# Autodesk Inventor assembly: Full overlay hinge for aluminium frame
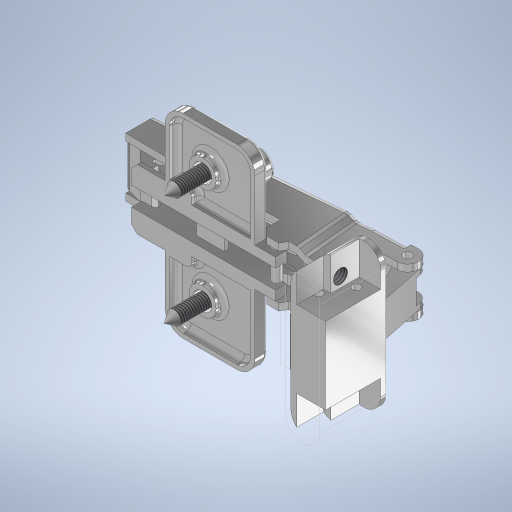
[picture p0: Inventor's stored thumbnail of the model, 512x512]
Saved by Autodesk Inventor 2024 (Build 280153000, 153)
## iProperties
Created: 2014-01-06
Part Number: Full overlay hinge for aluminium frame
Document SubType Name: Assembly
Designer: G. Kazokaitis
Author: G. Kazokaitis
## Documents named in this file (15)
- C:\W4INV 2024 Design\LIBRARY\Hinges\HINGE FOR ALUMINIUM FRAME.iam
- C:\W4INV 2024 Design\LIBRARY\Hinges\Parts\Hinge for aluminium frame\Full overlay case .ipt
- C:\W4INV 2024 Design\LIBRARY\Hinges\Parts\Hinge for aluminium frame\Lever for full overlay hinge.ipt
- C:\W4INV 2024 Design\LIBRARY\Hinges\Parts\Hinge for aluminium frame\Linkage for full overlay hinge.ipt
- C:\W4INV 2024 Design\LIBRARY\Hinges\Parts\Hinge for aluminium frame\Half overlay case.ipt
- C:\W4INV 2024 Design\LIBRARY\Hinges\Parts\Hinge for aluminium frame\Lever for half overlay hinge.ipt
- C:\W4INV 2024 Design\LIBRARY\Hinges\Parts\Hinge for aluminium frame\Linkage for half overlay hinge.ipt
- C:\W4INV 2024 Design\LIBRARY\Hinges\Parts\Hinge for aluminium frame\Inset case.ipt
- C:\W4INV 2024 Design\LIBRARY\Hinges\Parts\Hinge for aluminium frame\Lever for inset hinge.ipt
- C:\W4INV 2024 Design\LIBRARY\Hinges\Parts\Hinge for aluminium frame\Linkage for inset hinge.ipt
- C:\W4INV 2024 Design\LIBRARY\Hinges\Parts\Hinge for aluminium frame\Mounting plate.ipt
- C:\W4INV 2024 Design\LIBRARY\Hinges\Parts\Hinge for aluminium frame\Cup.ipt
- Full overlay hinge for aluminium frame.iam
- Half overlay hinge for aluminium frame.iam
- Inset hinge for aluminium frame.iam
## Components (11 placed, 11 different names)
1. Mounting plate:1 — Flush:1, Flush:2, Mate:1, Flush:3, Mate:2, Mate:3, Flush:4, Mate:11, Mate:12, Flush:5, Mate:20, Mate:21
2. Cup:1 — Mate:8, Mate:9, Mate:10, Full overlay opening angle, Mate:17, Mate:18, Mate:19, Half overlay opening angle, Mate:26, Mate:27, Mate:28, Inset hinge opening angle
3. Full overlay case :1 — Flush:3, Mate:2, Mate:3, Mate:4, Mate:5, Mate:6, Mate:7, Full overlay opening angle
4. Linkage for full overlay hinge:1 — Mate:5, Mate:7, Mate:9
5. Lever for full overlay hinge:1 — Mate:4, Mate:6, Mate:8, Mate:10
6. Half overlay case:1 — Flush:4, Mate:11, Mate:12, Mate:13, Mate:14, Mate:15, Mate:16, Half overlay opening angle
7. Lever for half overlay hinge:1 — Mate:13, Mate:14, Mate:17, Mate:19
8. Linkage for half overlay hinge:1 — Mate:15, Mate:16, Mate:18
9. Inset case:1 — Flush:5, Mate:20, Mate:21, Mate:22, Mate:23, Mate:24, Mate:25, Inset hinge opening angle
10. Lever for inset hinge:1 — Mate:22, Mate:23, Mate:26, Mate:28
11. Linkage for inset hinge:1 — Mate:24, Mate:25, Mate:27
## Relationships (36: Mate 28, Flush 5, Angle 3)
- Flush:1: Mounting plate:1
- Flush:2: Mounting plate:1
- Mate:1: Mounting plate:1
- Flush:3: Mounting plate:1 ↔ Full overlay case :1
- Mate:2: Mounting plate:1 ↔ Full overlay case :1
- Mate:3: Mounting plate:1 ↔ Full overlay case :1
- Mate:4: Full overlay case :1 ↔ Lever for full overlay hinge:1
- Mate:5: Full overlay case :1 ↔ Linkage for full overlay hinge:1
- Mate:6 (0.2 mm): Full overlay case :1 ↔ Lever for full overlay hinge:1
- Mate:7 (0.2 mm): Full overlay case :1 ↔ Linkage for full overlay hinge:1
- Mate:8: Cup:1 ↔ Lever for full overlay hinge:1
- Mate:9: Cup:1 ↔ Linkage for full overlay hinge:1
- Mate:10 (1.9 mm): Cup:1 ↔ Lever for full overlay hinge:1
- Full overlay opening angle [Angle] (180 deg): Cup:1 ↔ Full overlay case :1
- Flush:4: Mounting plate:1 ↔ Half overlay case:1
- Mate:11: Mounting plate:1 ↔ Half overlay case:1
- Mate:12: Mounting plate:1 ↔ Half overlay case:1
- Mate:13: Half overlay case:1 ↔ Lever for half overlay hinge:1
- Mate:14: Half overlay case:1 ↔ Lever for half overlay hinge:1
- Mate:15: Half overlay case:1 ↔ Linkage for half overlay hinge:1
- Mate:16: Half overlay case:1 ↔ Linkage for half overlay hinge:1
- Mate:17: Cup:1 ↔ Lever for half overlay hinge:1
- Mate:18: Cup:1 ↔ Linkage for half overlay hinge:1
- Mate:19 (1.9 mm): Cup:1 ↔ Lever for half overlay hinge:1
- Half overlay opening angle [Angle] (180 deg): Cup:1 ↔ Half overlay case:1
- Flush:5: Mounting plate:1 ↔ Inset case:1
- Mate:20: Mounting plate:1 ↔ Inset case:1
- Mate:21: Mounting plate:1 ↔ Inset case:1
- Mate:22: Inset case:1 ↔ Lever for inset hinge:1
- Mate:23: Inset case:1 ↔ Lever for inset hinge:1
- Mate:24: Inset case:1 ↔ Linkage for inset hinge:1
- Mate:25: Inset case:1 ↔ Linkage for inset hinge:1
- Mate:26: Cup:1 ↔ Lever for inset hinge:1
- Mate:27: Cup:1 ↔ Linkage for inset hinge:1
- Mate:28 (1.9 mm): Cup:1 ↔ Lever for inset hinge:1
- Inset hinge opening angle [Angle] (180 deg): Cup:1 ↔ Inset case:1
## Named parameters: Offset_distance = 37 mm
